# Autodesk Inventor assembly: tester
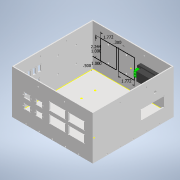
[picture p0: Inventor's stored thumbnail of the model, 180x180]
Saved by Autodesk Inventor 2020.2 (Build 242310000, 310)
## iProperties
Created: 2020-02-06
Part Number: tester
Document SubType Name: Assembly
Designer: ColinP
Author: ColinP
## Documents named in this file (8)
- C:\Users\ColinP\Documents\Inventor\HeaterControlIQC\sheetmetalversion2.0\tester.iam
- C:\Users\ColinP\Documents\Inventor\HeaterControlIQC\sheetmetalversion2.0\sheetmetalback2.0.ipt
- C:\Users\ColinP\Documents\Inventor\HeaterControlIQC\components\CUI_VSK-S5-5UA-T (1)\CUI_VSK-S5-5UA-T.iam
- C:\Users\ColinP\Documents\Inventor\HeaterControlIQC\sheetmetalversion2.0\sheetmetalbottom2.0.ipt
- C:\Users\ColinP\Documents\Inventor\HeaterControlIQC\sheetmetalversion2.0\sheetmetalface2.0.ipt
- C:\Users\ColinP\Documents\Inventor\HeaterControlIQC\sheetmetalversion2.0\sheetmetalleft2.0.ipt
- C:\Users\ColinP\Documents\Inventor\HeaterControlIQC\sheetmetalversion2.0\sheetmetalright2.0.ipt
- C:\Users\ColinP\Documents\Inventor\HeaterControlIQC\sheetmetalversion2.0\sheetmetaltop2.0.ipt
## Components (7 placed, 7 different names)
1. sheetmetalback2.0:1 — Mate:4, Mate:5, Mate:6, Mate:23, Mate:24, Mate:25
2. CUI_VSK-S5-5UA-T:1 [sub-assembly] — Mate:23, Mate:24, Mate:25
3. sheetmetalbottom2.0:1 — Mate:4, Mate:5, Mate:6, Mate:10, Mate:11, Mate:12, Mate:13, Mate:14, Mate:15, Mate:17, Mate:18, Mate:19
4. sheetmetalface2.0:1 — Mate:10, Mate:11, Mate:12
5. sheetmetalleft2.0:1 — Mate:17, Mate:18, Mate:19, Mate:22
6. sheetmetalright2.0:1 — Mate:13, Mate:14, Mate:15, Mate:16
7. sheetmetaltop2.0:1 — Mate:16, Mate:22
## Relationships (17: Mate 17)
- Mate:4: sheetmetalback2.0:1 ↔ sheetmetalbottom2.0:1
- Mate:5: sheetmetalback2.0:1 ↔ sheetmetalbottom2.0:1
- Mate:6: sheetmetalback2.0:1 ↔ sheetmetalbottom2.0:1
- Mate:10: sheetmetalbottom2.0:1 ↔ sheetmetalface2.0:1
- Mate:11: sheetmetalbottom2.0:1 ↔ sheetmetalface2.0:1
- Mate:12: sheetmetalbottom2.0:1 ↔ sheetmetalface2.0:1
- Mate:13: sheetmetalbottom2.0:1 ↔ sheetmetalright2.0:1
- Mate:14: sheetmetalbottom2.0:1 ↔ sheetmetalright2.0:1
- Mate:15: sheetmetalbottom2.0:1 ↔ sheetmetalright2.0:1
- Mate:16: sheetmetalright2.0:1 ↔ sheetmetaltop2.0:1
- Mate:17: sheetmetalbottom2.0:1 ↔ sheetmetalleft2.0:1
- Mate:18: sheetmetalbottom2.0:1 ↔ sheetmetalleft2.0:1
- Mate:19: sheetmetalbottom2.0:1 ↔ sheetmetalleft2.0:1
- Mate:22: sheetmetalleft2.0:1 ↔ sheetmetaltop2.0:1
- Mate:23: sheetmetalback2.0:1 ↔ CUI_VSK-S5-5UA-T:1
- Mate:24: sheetmetalback2.0:1 ↔ CUI_VSK-S5-5UA-T:1
- Mate:25: sheetmetalback2.0:1 ↔ CUI_VSK-S5-5UA-T:1
